# Autodesk Inventor assembly: Auto
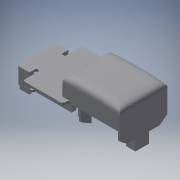
[picture p0: Inventor's stored thumbnail of the model, 180x180]
Saved by Autodesk Inventor 2018.3 (Build 223284000, 284)
## iProperties
Created: 2018-08-17
Part Number: Auto
Material: Generisch
Document SubType Name: Assembly
## Documents named in this file (4)
- U:\COSIMA-Laserstar\CAD\Auto.iam
- U:\COSIMA-Laserstar\CAD\Platte Auto.ipt
- U:\COSIMA-Laserstar\CAD\files\arduino-uno-r3-1.snapshot.3\arduino uno.iam
- C:\Users\PRYADUN\Documents\Deckel.ipt
## Components (3 placed, 3 different names)
1. Platte Auto:1 — Winkel:1, Passend:1, Winkel:2, Passend:2, Passend:3, Fluchtend:1, Fluchtend:2
2. arduino uno:1 [sub-assembly] — Winkel:1, Passend:1, Winkel:2, Passend:2, Passend:3
3. Deckel:1 — Fluchtend:1, Fluchtend:2
## Relationships (7: Mate 3, Angle 2, Flush 2)
- Winkel:1 [Angle] (180 deg): Platte Auto:1 ↔ arduino uno:1
- Passend:1 [Mate]: Platte Auto:1 ↔ arduino uno:1
- Winkel:2 [Angle] (0 deg): Platte Auto:1 ↔ arduino uno:1
- Passend:2 [Mate] (-26.67 mm): Platte Auto:1 ↔ arduino uno:1
- Passend:3 [Mate] (10 mm): Platte Auto:1 ↔ arduino uno:1
- Fluchtend:1 [Flush]: Platte Auto:1 ↔ Deckel:1
- Fluchtend:2 [Flush]: Platte Auto:1 ↔ Deckel:1
